# Autodesk Inventor assembly: czlon i przekladnia
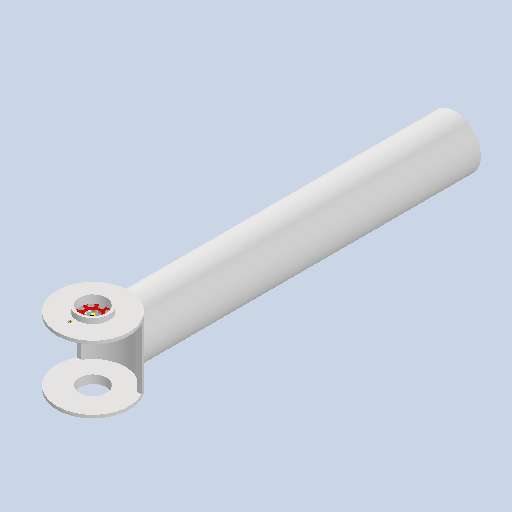
[picture p0: Inventor's stored thumbnail of the model, 512x512]
Saved by Autodesk Inventor 2023 (Build 270158000, 158)
## iProperties
Created: 2023-04-08
Part Number: czlon i przekladnia
Document SubType Name: Assembly
Designer: Wiktor
Author: Wiktor
## Documents named in this file (4)
- C:\Users\Wiktor\Documents\Manipulator\czlon i przekladnia.iam
- C:\Users\Wiktor\Documents\Manipulator\czlon_1.ipt
- C:\Users\Wiktor\Documents\Manipulator\Przekładnia cykloidalna mimośrodowa.ipt
- C:\Users\Wiktor\Documents\Manipulator\Przekładnia rolka.ipt
## Components (3 placed, 3 different names)
1. czlon_1:1 — Zestawiające:4, Zestawiające:5, Zestawiające:7
2. Przekładnia cykloidalna mimośrodowa:1 — Zestawiające:3, Styczny:1, Zestawiające:4, Zestawiające:5
3. Przekładnia rolka:1 — Zestawiające:3, Styczny:1, Zestawiające:6
## Relationships (7: Mate 6, Tangent 1)
- Zestawiające:3 [Mate]: Przekładnia cykloidalna mimośrodowa:1 ↔ Przekładnia rolka:1
- Styczny:1 [Tangent]: Przekładnia cykloidalna mimośrodowa:1 ↔ Przekładnia rolka:1
- Zestawiające:4 [Mate]: czlon_1:1 ↔ Przekładnia cykloidalna mimośrodowa:1
- Zestawiające:5 [Mate]: czlon_1:1 ↔ Przekładnia cykloidalna mimośrodowa:1
- Zestawiające:6 [Mate]: Przekładnia rolka:1
- Zestawiające:7 [Mate]: czlon_1:1
- Zestawiające:8 [Mate]
